# Autodesk Inventor assembly: Assembly2
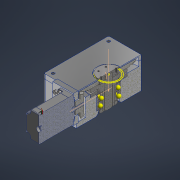
[picture p0: Inventor's stored thumbnail of the model, 180x180]
Saved by Autodesk Inventor 2022 (Build 260153000, 153)
## iProperties
Part Number: Assembly2
Document SubType Name: Assembly
Designer: Andres
Author: Andres
## Documents named in this file (19)
- D:\Documentos\15.PUCP_2021-2\[PDM] Proyecto de Diseño Mecatrónico\ProyectoGIT\ProyectoRobotPallet\SistemaDeElevacion\version2\Assembly2.iam
- SistemaElevacion2.iam
- D:\Documentos\15.PUCP_2021-2\[PDM] Proyecto de Diseño Mecatrónico\ProyectoGIT\ProyectoRobotPallet\SistemaDeElevacion\version2\Soporte.ipt
- D:\Documentos\15.PUCP_2021-2\[PDM] Proyecto de Diseño Mecatrónico\ProyectoGIT\ProyectoRobotPallet\SistemaDeElevacion\version2\Tuerca3.ipt
- D:\Documentos\15.PUCP_2021-2\[PDM] Proyecto de Diseño Mecatrónico\ProyectoGIT\ProyectoRobotPallet\SistemaDeElevacion\AIS2021\SKF_7205 BE-2RZP.iam
- D:\Documentos\15.PUCP_2021-2\[PDM] Proyecto de Diseño Mecatrónico\ProyectoGIT\ProyectoRobotPallet\SistemaDeElevacion\version2\Assembly2\Design Accelerator\Bevel Gears3.iam
- D:\Documentos\15.PUCP_2021-2\[PDM] Proyecto de Diseño Mecatrónico\ProyectoGIT\ProyectoRobotPallet\SistemaDeElevacion\version2\SeguroRodamientos.ipt
- D:\Documentos\15.PUCP_2021-2\[PDM] Proyecto de Diseño Mecatrónico\ProyectoGIT\ProyectoRobotPallet\SistemaDeElevacion\Tornillo de elevación.ipt
- D:\Documentos\15.PUCP_2021-2\[PDM] Proyecto de Diseño Mecatrónico\ProyectoGIT\ProyectoRobotPallet\SistemaDeElevacion\SKF_MB 5.ipt
- D:\Documentos\15.PUCP_2021-2\[PDM] Proyecto de Diseño Mecatrónico\ProyectoGIT\ProyectoRobotPallet\SistemaDeElevacion\SKF_KM 5.ipt
- D:\Documentos\15.PUCP_2021-2\[PDM] Proyecto de Diseño Mecatrónico\ProyectoGIT\ProyectoRobotPallet\Tapa.ipt
- D:\Documentos\15.PUCP_2021-2\[PDM] Proyecto de Diseño Mecatrónico\ProyectoGIT\ProyectoRobotPallet\MonturaMotor.ipt
- D:\Documentos\15.PUCP_2021-2\[PDM] Proyecto de Diseño Mecatrónico\ProyectoGIT\ProyectoRobotPallet\SistemaDeElevacion\NEMA 23 - 76mm.ipt
- D:\Documentos\15.PUCP_2021-2\[PDM] Proyecto de Diseño Mecatrónico\ProyectoGIT\ProyectoRobotPallet\ContentCenter\en-US\ISO 4762(2)\ISO 4762 - M4 x 16ISO.ipt
- D:\Documentos\15.PUCP_2021-2\[PDM] Proyecto de Diseño Mecatrónico\ProyectoGIT\ProyectoRobotPallet\ContentCenter\en-US\ISO 4762(2)\ISO 4762 - M4 x 12ISO.ipt
- D:\Documentos\15.PUCP_2021-2\[PDM] Proyecto de Diseño Mecatrónico\ProyectoGIT\ProyectoRobotPallet\ContentCenter\en-US\ISO 4762(2)\ISO 4762 - M4 x 10ISO.ipt
- D:\Documentos\15.PUCP_2021-2\[PDM] Proyecto de Diseño Mecatrónico\ProyectoGIT\ProyectoRobotPallet\ContentCenter\en-US\ISO 4762(2)\ISO 4762 - M3 x 10ISO.ipt
- D:\Documentos\15.PUCP_2021-2\[PDM] Proyecto de Diseño Mecatrónico\ProyectoGIT\ProyectoRobotPallet\BridaTornillo2.ipt
- D:\Documentos\15.PUCP_2021-2\[PDM] Proyecto de Diseño Mecatrónico\ProyectoGIT\ProyectoRobotPallet\ContentCenter\en-US\ISO 4762(2)\ISO 4762 - M3 x 12ISO.ipt
## Components (37 placed, 17 different names)
1. Soporte:1 — Flush:1, Mate:3, Mate:4, Flush:2, Mate:10, Mate:11, Flush:3, Flush:4, Mate:17, Angle:4
2. Tuerca3:1 — Flush:1, Mate:12, Mate:15, Mate:16, Angle:1, Mate:21
3. SKF_7205 BE-2RZP:1 [sub-assembly] — Mate:1, Mate:2, Mate:3, Mate:4
4. SKF_7205 BE-2RZP:2 [sub-assembly] — Mate:1, Mate:2
5. Bevel Gears:1 [sub-assembly] — Mate:16, Angle:1, Mate:17, Mate:18, Insert:9, Insert:10, Insert:11, Insert:12, Insert:13, Insert:14
6. SeguroRodamientos:1 — Flush:2, Mate:10, Mate:11, Insert:15, Insert:16, Insert:17, Insert:18, Insert:19, Insert:20
7. Tornillo de elevación:1 — Mate:12, Flush:5, Flush:6, Mate:20, Angle:3, Angle:4
8. SKF_MB 5:1 — Mate:13, Mate:14
9. SKF_KM 5:1 — Mate:13, Mate:14, Mate:15
10. Tapa:1 — Flush:3, Insert:21, Insert:22, Insert:23, Insert:24
11. MonturaMotor:1 — Flush:4, Angle:2, Insert:1, Insert:2, Insert:3, Insert:4, Mate:19
12. NEMA 23 - 76mm:1 — Mate:18, Angle:2, Insert:5, Insert:6, Insert:7, Insert:8, Mate:19
13. ISO 4762 M4 x 16:1 — Insert:1
14. ISO 4762 M4 x 16:2 — Insert:2
15. ISO 4762 M4 x 16:3 — Insert:3
16. ISO 4762 M4 x 16:4 — Insert:4
17. ISO 4762 M4 x 12:1 — Insert:5
18. ISO 4762 M4 x 12:2 — Insert:6
19. ISO 4762 M4 x 12:3 — Insert:7
20. ISO 4762 M4 x 12:4 — Insert:8
21. ISO 4762 M4 x 10:1 — Insert:9
22. ISO 4762 M4 x 10:2 — Insert:10
23. ISO 4762 M4 x 10:3 — Insert:11
24. ISO 4762 M4 x 10:4 — Insert:12
25. ISO 4762 M4 x 10:5 — Insert:13
26. ISO 4762 M4 x 10:6 — Insert:14
27. ISO 4762 M3 x 10:1 — Insert:15
28. ISO 4762 M3 x 10:2 — Insert:16
29. ISO 4762 M3 x 10:3 — Insert:17
30. ISO 4762 M3 x 10:4 — Insert:18
31. ISO 4762 M3 x 10:5 — Insert:19
32. ISO 4762 M3 x 10:6 — Insert:20
33. BridaTornillo2:1 — Flush:5, Flush:6, Mate:20, Angle:3, Mate:21
34. ISO 4762 M3 x 12:1 — Insert:21
35. ISO 4762 M3 x 12:2 — Insert:22
36. ISO 4762 M3 x 12:3 — Insert:23
37. ISO 4762 M3 x 12:4 — Insert:24
## Relationships (50: Insert 24, Mate 16, Flush 6, Angle 4)
- Flush:1: Soporte:1 ↔ Tuerca3:1
- Mate:1: SKF_7205 BE-2RZP:1 ↔ SKF_7205 BE-2RZP:2
- Mate:2: SKF_7205 BE-2RZP:1 ↔ SKF_7205 BE-2RZP:2
- Mate:3: Soporte:1 ↔ SKF_7205 BE-2RZP:1
- Mate:4: Soporte:1 ↔ SKF_7205 BE-2RZP:1
- Flush:2: Soporte:1 ↔ SeguroRodamientos:1
- Mate:10: Soporte:1 ↔ SeguroRodamientos:1
- Mate:11: Soporte:1 ↔ SeguroRodamientos:1
- Mate:12: Tuerca3:1 ↔ Tornillo de elevación:1
- Mate:13: SKF_MB 5:1 ↔ SKF_KM 5:1
- Mate:14: SKF_MB 5:1 ↔ SKF_KM 5:1
- Mate:15: Tuerca3:1 ↔ SKF_KM 5:1
- Flush:3: Soporte:1 ↔ Tapa:1
- Flush:4: Soporte:1 ↔ MonturaMotor:1
- Mate:16: Tuerca3:1 ↔ Bevel Gears:1
- Angle:1 (0 deg): Tuerca3:1 ↔ Bevel Gears:1
- Mate:17: Soporte:1 ↔ Bevel Gears:1
- Mate:18: Bevel Gears:1 ↔ NEMA 23 - 76mm:1
- Angle:2 (0 deg): MonturaMotor:1 ↔ NEMA 23 - 76mm:1
- Insert:1: MonturaMotor:1 ↔ ISO 4762 M4 x 16:1
- Insert:2: MonturaMotor:1 ↔ ISO 4762 M4 x 16:2
- Insert:3: MonturaMotor:1 ↔ ISO 4762 M4 x 16:3
- Insert:4: MonturaMotor:1 ↔ ISO 4762 M4 x 16:4
- Insert:5: NEMA 23 - 76mm:1 ↔ ISO 4762 M4 x 12:1
- Insert:6: NEMA 23 - 76mm:1 ↔ ISO 4762 M4 x 12:2
- Insert:7: NEMA 23 - 76mm:1 ↔ ISO 4762 M4 x 12:3
- Insert:8: NEMA 23 - 76mm:1 ↔ ISO 4762 M4 x 12:4
- Mate:19: MonturaMotor:1 ↔ NEMA 23 - 76mm:1
- Insert:9: Bevel Gears:1 ↔ ISO 4762 M4 x 10:1
- Insert:10: Bevel Gears:1 ↔ ISO 4762 M4 x 10:2
- Insert:11: Bevel Gears:1 ↔ ISO 4762 M4 x 10:3
- Insert:12: Bevel Gears:1 ↔ ISO 4762 M4 x 10:4
- Insert:13: Bevel Gears:1 ↔ ISO 4762 M4 x 10:5
- Insert:14: Bevel Gears:1 ↔ ISO 4762 M4 x 10:6
- Insert:15: SeguroRodamientos:1 ↔ ISO 4762 M3 x 10:1
- Insert:16: SeguroRodamientos:1 ↔ ISO 4762 M3 x 10:2
- Insert:17: SeguroRodamientos:1 ↔ ISO 4762 M3 x 10:3
- Insert:18: SeguroRodamientos:1 ↔ ISO 4762 M3 x 10:4
- Insert:19: SeguroRodamientos:1 ↔ ISO 4762 M3 x 10:5
- Insert:20: SeguroRodamientos:1 ↔ ISO 4762 M3 x 10:6
- Flush:5: Tornillo de elevación:1 ↔ BridaTornillo2:1
- Flush:6: Tornillo de elevación:1 ↔ BridaTornillo2:1
- Mate:20: Tornillo de elevación:1 ↔ BridaTornillo2:1
- Angle:3 (0 deg): Tornillo de elevación:1 ↔ BridaTornillo2:1
- Angle:4 (0 deg): Soporte:1 ↔ Tornillo de elevación:1
- Mate:21: Tuerca3:1 ↔ BridaTornillo2:1
- Insert:21: Tapa:1 ↔ ISO 4762 M3 x 12:1
- Insert:22: Tapa:1 ↔ ISO 4762 M3 x 12:2
- Insert:23: Tapa:1 ↔ ISO 4762 M3 x 12:3
- Insert:24: Tapa:1 ↔ ISO 4762 M3 x 12:4
